# Autodesk Inventor assembly: battery-stopper-assembly-multiple
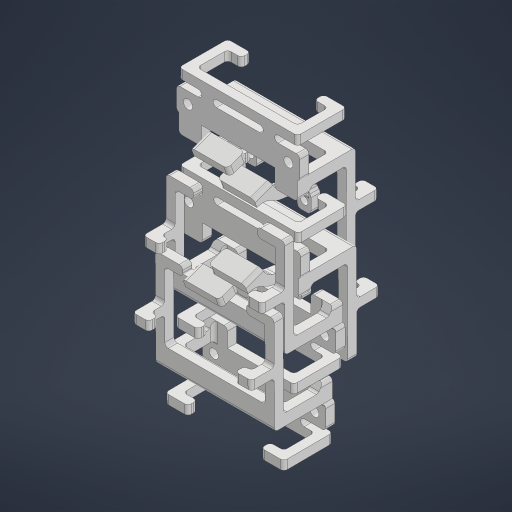
[picture p0: Inventor's stored thumbnail of the model, 512x512]
Saved by Autodesk Inventor 2023.5 (Build 275446000, 446)
## iProperties
Created: 2025-02-09
Part Number: battery-stopper-assembly-multiple
Document SubType Name: Assembly
Designer: IshiiLabHonda
Author: IshiiLabHonda
## Documents named in this file (4)
- C:\Users\IshiiLabHonda\Documents\Micromouse\Passion-v2\Inventor\Passion-v2-6\DMM\battery-stopper-assembly-multiple.iam
- C:\Users\IshiiLabHonda\Documents\Micromouse\Passion-v2\Inventor\Passion-v2-6\DMM\battery-stopper-3\battery-stopper-3.ipt
- C:\Users\IshiiLabHonda\Documents\Micromouse\Passion-v2\Inventor\Passion-v2-6\DMM\battery-stopper-1\battery-stopper-1.ipt
- C:\Users\IshiiLabHonda\Documents\Micromouse\Passion-v2\Inventor\Passion-v2-6\DMM\battery-stopper-1-mirror\battery-stopper-1-mirror.ipt
## Components (8 placed, 3 different names)
1. battery-stopper-3:1 — メイト:1
2. battery-stopper-1:1
3. battery-stopper-1-mirror:1
4. battery-stopper-3:2
5. battery-stopper-3:3
6. battery-stopper-1:2
7. battery-stopper-1-mirror:2
8. battery-stopper-3:4
## Relationships (1: Mate 1)
- メイト:1 [Mate]: battery-stopper-3:1
